# Autodesk Inventor assembly: estação_bga
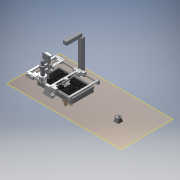
[picture p0: Inventor's stored thumbnail of the model, 180x180]
Saved by Autodesk Inventor 2018 (Build 220112000, 112)
## iProperties
Created: 2018-05-03
Part Number: estação_bga
Material: Genérico
Document SubType Name: Assembly
Designer: Georgines
Author: Georgines
## Documents named in this file (8)
- C:\Users\Georgines\Downloads\pecas_3d-20180530T120808Z-001\pecas_3d\estacao.iam
- C:\Users\Georgines\Downloads\pecas_3d-20180530T120808Z-001\pecas_3d\mesa_aquecimento.iam
- C:\Users\Georgines\Downloads\pecas_3d-20180530T120808Z-001\pecas_3d\mesa_suporte_de_placa.iam
- C:\Users\Georgines\Downloads\pecas_3d-20180530T120808Z-001\pecas_3d\cabeça_inferior.iam
- C:\Users\Georgines\Downloads\pecas_3d-20180530T120808Z-001\pecas_3d\cabeça_superior.iam
- C:\Users\Georgines\Downloads\pecas_3d-20180530T120808Z-001\pecas_3d\bocal_inferior.ipt
- C:\Users\Georgines\Downloads\pecas_3d-20180530T120808Z-001\pecas_3d\braço_junta_1.ipt
- C:\Users\Georgines\Downloads\pecas_3d-20180530T120808Z-001\pecas_3d\braço_junta_2.ipt
## Components (8 placed, 7 different names)
1. mesa_aquecimento:1 [sub-assembly] — Coincidência:1, Coincidência:2, Coincidência:4, Coincidência:5
2. mesa_suporte_de_placa:1 [sub-assembly] — Coincidência:3, Ângulo:1
3. cabeça_inferior:1 [sub-assembly] — Coincidência:4, Coincidência:5, Coincidência:6, Coincidência:7, Ângulo:1
4. bocal_inferior:1 — Coincidência:6, Coincidência:7
5. bocal_inferior:2
6. braço_junta_1:1 — Alinhamento:1
7. braço_junta_2:1 — Coincidência:8, Alinhamento:2
8. cabeça_superior:1 [sub-assembly] — Coincidência:8, Alinhamento:2
## Relationships (11: Mate 8, Flush 2, Angle 1)
- Coincidência:1 [Mate]: mesa_aquecimento:1
- Coincidência:2 [Mate]: mesa_aquecimento:1
- Coincidência:3 [Mate]: mesa_suporte_de_placa:1
- Coincidência:4 [Mate]: mesa_aquecimento:1 ↔ cabeça_inferior:1
- Coincidência:5 [Mate]: mesa_aquecimento:1 ↔ cabeça_inferior:1
- Coincidência:6 [Mate]: cabeça_inferior:1 ↔ bocal_inferior:1
- Coincidência:7 [Mate]: cabeça_inferior:1 ↔ bocal_inferior:1
- Ângulo:1 [Angle] (0 deg): mesa_suporte_de_placa:1 ↔ cabeça_inferior:1
- Alinhamento:1 [Flush]: braço_junta_1:1
- Coincidência:8 [Mate]: braço_junta_2:1 ↔ cabeça_superior:1
- Alinhamento:2 [Flush] (10 mm): braço_junta_2:1 ↔ cabeça_superior:1
